# Autodesk Inventor assembly: Draft_02_Assembly
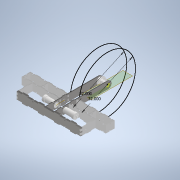
[picture p0: Inventor's stored thumbnail of the model, 180x180]
Saved by Autodesk Inventor 2021 (Build 250183000, 183)
## iProperties
Created: 2021-03-08
Part Number: Draft_02_Assembly
Document SubType Name: Assembly
Designer: M3rob
Mass: 43980.5 g
Surface Area: 13842.3 cm^2
Volume: 8165.67 cm^3
Density: 5.38602 g/cm^3
Author: M3rob
## Documents named in this file (11)
- C:\Users\M3rob\Documents\GrabCAD\FireBird 250 Pound Gaming Machine\Drafts\FrameDrafts\Draft_02\Draft_02_Assembly.iam
- C:\Users\M3rob\Documents\GrabCAD\FireBird 250 Pound Gaming Machine\Drafts\FrameDrafts\Draft_02\NeckFrame_02.ipt
- C:\Users\M3rob\Documents\GrabCAD\FireBird 250 Pound Gaming Machine\Drafts\FrameDrafts\Draft_02\BackWallFrame_02.ipt
- C:\Users\M3rob\Documents\GrabCAD\FireBird 250 Pound Gaming Machine\Drafts\FrameDrafts\Draft_02\DriveSideFrame_02.ipt
- C:\Users\M3rob\Documents\GrabCAD\FireBird 250 Pound Gaming Machine\Drafts\FrameDrafts\Draft_02\FrontWallFrame_02.ipt
- C:\Users\M3rob\Documents\GrabCAD\FireBird 250 Pound Gaming Machine\Drafts\FrameDrafts\Draft_02\SmallSideFrame_02.ipt
- C:\Users\M3rob\Documents\GrabCAD\FireBird 250 Pound Gaming Machine\Drafts\FrameDrafts\Draft_02\weeeeapon.ipt
- C:\Users\M3rob\Documents\GrabCAD\FireBird 250 Pound Gaming Machine\Drafts\FrameDrafts\Draft_02\Draft_02_Assembly\Design Accelerator\Bearing4.iam
- C:\Users\M3rob\Documents\GrabCAD\FireBird 250 Pound Gaming Machine\Drafts\FrameDrafts\Draft_02\WeaponHub.ipt
- C:\Users\M3rob\Documents\GrabCAD\FireBird 250 Pound Gaming Machine\Drafts\FrameDrafts\Draft_02\Draft_02_Assembly\Design Accelerator\Bearing5.iam
- C:\Users\M3rob\Documents\GrabCAD\FireBird 250 Pound Gaming Machine\MotorMockup.ipt
## Components (21 placed, 9 different names)
1. NeckFrame_02:1 — Flush:1, Flush:2, Mate:1, Mate:2, Mate:4, Mate:8, Flush:6, Flush:7, Flush:13, Flush:14, Mate:11, Mate:35, Flush:37, Mate:38, Mate:45, Mate:48, Flush:38
2. NeckFrame_02:2 — Flush:1, Flush:2, Mate:3, Mate:9, Flush:8, Flush:9, Mate:10, Flush:10, Flush:11, Mate:27, Mate:34, Flush:36, Mate:37, Mate:49, Flush:39
3. BackWallFrame_02:1 — Mate:1, Mate:2, Mate:3, Mate:4, Mate:5, Flush:3, Mate:6, Mate:7, Flush:4, Flush:5
4. DriveSideFrame_02:1 — Mate:5, Flush:3, Mate:6
5. DriveSideFrame_02:2 — Mate:7, Flush:4, Flush:5
6. FrontWallFrame_02:1 — Mate:10, Flush:10, Flush:11, Mate:16, Mate:17, Flush:17, Mate:18, Mate:19
7. FrontWallFrame_02:2 — Mate:9, Flush:8, Flush:9, Flush:18, Flush:19
8. FrontWallFrame_02:3 — Mate:8, Flush:6, Flush:7, Flush:16
9. FrontWallFrame_02:4 — Flush:13, Flush:14, Mate:11, Mate:12, Mate:13, Flush:15, Mate:14, Mate:15
10. SmallSideFrame_02:1 — Mate:18, Mate:19, Flush:18
11. SmallSideFrame_02:2 — Mate:16, Mate:17, Flush:17, Flush:19
12. SmallSideFrame_02:3 — Mate:14, Mate:15, Flush:16
13. SmallSideFrame_02:4 — Mate:12, Mate:13, Flush:15
14. weeeeapon:1 — Mate:36, Mate:39, Mate:40
15. Bearing:4 [sub-assembly] — Mate:34, Flush:36
16. Bearing:5 [sub-assembly] — Mate:35, Flush:37
17. WeaponHub:1 — Mate:36, Mate:37, Mate:38, Mate:39, Mate:40, Mate:41, Mate:42, Mate:43, Mate:44
18. Bearing:6 [sub-assembly] — Mate:41, Mate:44
19. Bearing:7 [sub-assembly] — Mate:42, Mate:43
20. MotorMockup:1 — Mate:48, Flush:38
21. MotorMockup:2 — Mate:49, Flush:39
## Relationships (59: Mate 37, Flush 22)
- Flush:1: NeckFrame_02:1 ↔ NeckFrame_02:2
- Flush:2: NeckFrame_02:1 ↔ NeckFrame_02:2
- Mate:1: NeckFrame_02:1 ↔ BackWallFrame_02:1
- Mate:2: NeckFrame_02:1 ↔ BackWallFrame_02:1
- Mate:3: NeckFrame_02:2 ↔ BackWallFrame_02:1
- Mate:4: NeckFrame_02:1 ↔ BackWallFrame_02:1
- Mate:5: BackWallFrame_02:1 ↔ DriveSideFrame_02:1
- Flush:3: BackWallFrame_02:1 ↔ DriveSideFrame_02:1
- Mate:6: BackWallFrame_02:1 ↔ DriveSideFrame_02:1
- Mate:7: BackWallFrame_02:1 ↔ DriveSideFrame_02:2
- Flush:4: BackWallFrame_02:1 ↔ DriveSideFrame_02:2
- Flush:5: BackWallFrame_02:1 ↔ DriveSideFrame_02:2
- Mate:8: NeckFrame_02:1 ↔ FrontWallFrame_02:3
- Flush:6: NeckFrame_02:1 ↔ FrontWallFrame_02:3
- Flush:7: NeckFrame_02:1 ↔ FrontWallFrame_02:3
- Mate:9: NeckFrame_02:2 ↔ FrontWallFrame_02:2
- Flush:8: NeckFrame_02:2 ↔ FrontWallFrame_02:2
- Flush:9: NeckFrame_02:2 ↔ FrontWallFrame_02:2
- Mate:10: NeckFrame_02:2 ↔ FrontWallFrame_02:1
- Flush:10: NeckFrame_02:2 ↔ FrontWallFrame_02:1
- Flush:11: NeckFrame_02:2 ↔ FrontWallFrame_02:1
- Flush:13: NeckFrame_02:1 ↔ FrontWallFrame_02:4
- Flush:14: NeckFrame_02:1 ↔ FrontWallFrame_02:4
- Mate:11: NeckFrame_02:1 ↔ FrontWallFrame_02:4
- Mate:12: FrontWallFrame_02:4 ↔ SmallSideFrame_02:4
- Mate:13: FrontWallFrame_02:4 ↔ SmallSideFrame_02:4
- Flush:15: FrontWallFrame_02:4 ↔ SmallSideFrame_02:4
- Mate:14: FrontWallFrame_02:4 ↔ SmallSideFrame_02:3
- Mate:15: FrontWallFrame_02:4 ↔ SmallSideFrame_02:3
- Flush:16: FrontWallFrame_02:3 ↔ SmallSideFrame_02:3
- Mate:16: FrontWallFrame_02:1 ↔ SmallSideFrame_02:2
- Mate:17: FrontWallFrame_02:1 ↔ SmallSideFrame_02:2
- Flush:17: FrontWallFrame_02:1 ↔ SmallSideFrame_02:2
- Mate:18: FrontWallFrame_02:1 ↔ SmallSideFrame_02:1
- Mate:19: FrontWallFrame_02:1 ↔ SmallSideFrame_02:1
- Flush:18: FrontWallFrame_02:2 ↔ SmallSideFrame_02:1
- Flush:19: FrontWallFrame_02:2 ↔ SmallSideFrame_02:2
- Mate:27: NeckFrame_02:2
- Mate:28
- Mate:29
- Mate:34: NeckFrame_02:2 ↔ Bearing:4
- Flush:36: NeckFrame_02:2 ↔ Bearing:4
- Mate:35: NeckFrame_02:1 ↔ Bearing:5
- Flush:37: NeckFrame_02:1 ↔ Bearing:5
- Mate:36: weeeeapon:1 ↔ WeaponHub:1
- Mate:37: NeckFrame_02:2 ↔ WeaponHub:1
- Mate:38 (3.175 mm): NeckFrame_02:1 ↔ WeaponHub:1
- Mate:39: weeeeapon:1 ↔ WeaponHub:1
- Mate:40: weeeeapon:1 ↔ WeaponHub:1
- Mate:41: WeaponHub:1 ↔ Bearing:6
- Mate:42: WeaponHub:1 ↔ Bearing:7
- Mate:43: WeaponHub:1 ↔ Bearing:7
- Mate:44: WeaponHub:1 ↔ Bearing:6
- Mate:45: NeckFrame_02:1
- Mate:47
- Mate:48: NeckFrame_02:1 ↔ MotorMockup:1
- Mate:49: NeckFrame_02:2 ↔ MotorMockup:2
- Flush:38: NeckFrame_02:1 ↔ MotorMockup:1
- Flush:39: NeckFrame_02:2 ↔ MotorMockup:2
